# Autodesk Inventor assembly: driver station
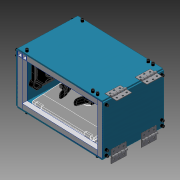
[picture p0: Inventor's stored thumbnail of the model, 180x180]
Saved by Autodesk Inventor 2015 (Build 190159000, 159)
## iProperties
Created: 2015-07-04
Part Number: driver station
Document SubType Name: Assembly
Designer: tsayman
Author: tsayman
## Documents named in this file (15)
- C:\Users\Owner\Documents\GrabCAD\Driver Station\driver station.iam
- C:\Users\Owner\Documents\GrabCAD\Driver Station\Part1.ipt
- C:\Users\Owner\Documents\GrabCAD\Driver Station\Part2.ipt
- C:\Users\Owner\Documents\GrabCAD\Driver Station\Part3.ipt
- C:\Users\Owner\Documents\GrabCAD\Driver Station\Part4.ipt
- C:\Users\Owner\Documents\GrabCAD\Driver Station\Part5.ipt
- C:\Users\Owner\Documents\GrabCAD\Driver Station\Imported Components\Assembly1.iam
- C:\Users\Owner\Documents\GrabCAD\Driver Station\Part6.ipt
- C:\Users\Owner\Documents\GrabCAD\Driver Station\Part7.ipt
- C:\Users\Owner\Documents\GrabCAD\Driver Station\Part8.ipt
- C:\Users\Owner\Documents\GrabCAD\Driver Station\buttonbox standin.ipt
- C:\Users\Owner\Documents\GrabCAD\Driver Station\logitech joystick.ipt
- C:\Users\Owner\Documents\GrabCAD\Driver Station\laptopstandin.ipt
- C:\Users\Owner\Documents\GrabCAD\Driver Station\finalhinge.ipt
- C:\Users\Owner\Documents\GrabCAD\Driver Station\bumper.ipt
## Components (46 placed, 20 different names)
1. bar1 — Mate:12, Flush:19, Flush:20
2. bar 2 — Flush:23, Mate:14, Flush:24
3. bar3 — Flush:21, Flush:22, Mate:13
4. bar4 — Mate:11, Flush:17, Flush:18
5. bar5 — Mate:9, Flush:12, Flush:13
6. bar6 — Mate:6, Flush:6, Flush:7
7. bar7 — Mate:8, Flush:10, Flush:11
8. bar8 — Flush:15, Mate:10, Flush:16
9. bar9 — Mate:3, Flush:4, Flush:14
10. bar10 — Mate:7, Flush:8, Flush:9
11. laptop asm [sub-assembly] — Mate:18
12. left panel — Mate:1, Flush:1, Mate:12, Flush:19, Flush:20, Flush:21, Flush:22, Mate:13, Flush:23, Mate:14, Flush:24, Mate:16, Flush:31, Flush:32, Angle:3, Flush:45, Flush:46, Mate:40, Mate:41, Mate:42, Mate:43, Mate:44, Mate:57, Mate:58, Mate:59, Mate:60, Mate:61
13. bottom pannel — Mate:1, Flush:1, Mate:2, Flush:3, Mate:3, Flush:4, Flush:14, Flush:15, Mate:10, Flush:16, Mate:17, Flush:33, Flush:34, Mate:18, Angle:1, Angle:3, Mate:23, Mate:24, Flush:35, Flush:36, Mate:36, Mate:38, Mate:39, Mate:55, Mate:56, Mate:64, Mate:65, Mate:66
14. top pannel — Flush:5, Mate:4, Mate:6, Flush:6, Flush:7, Mate:7, Flush:8, Flush:9, Mate:8, Flush:10, Flush:11, Rigid:2, Angle:2, Mate:19, Mate:20, Flush:39, Flush:40, Flush:41, Flush:42, Mate:25, Mate:26, Mate:27, Mate:28, Mate:29, Mate:30, Mate:45, Mate:46, Mate:47, Mate:48, Mate:49, Mate:50
15. right pannel — Mate:2, Flush:3, Flush:5, Mate:4, Mate:9, Flush:12, Flush:13, Mate:11, Flush:17, Flush:18, Rigid:1, Angle:1, Angle:2, Mate:21, Mate:22, Flush:37, Flush:38, Flush:43, Flush:44, Mate:31, Mate:32, Mate:33, Mate:34, Mate:35, Mate:51, Mate:52, Mate:53, Mate:54, Mate:62, Mate:63
16. buttonbox standin:1 — Rigid:2
17. logitech joystick:1 — Rigid:1
18. logitech joystick:2 — Mate:16, Flush:31, Flush:32
19. laptopstandin:1 — Mate:17, Flush:33, Flush:34
20. finalhinge:1 — Mate:19, Flush:40, Flush:42
21. finalhinge:2 — Mate:20, Flush:39, Flush:41
22. finalhinge:3 — Mate:22, Flush:38, Flush:43
23. finalhinge:4 — Mate:21, Flush:37, Flush:44
24. finalhinge:5 — Mate:24, Flush:36, Flush:45
25. finalhinge:6 — Mate:23, Flush:35, Flush:46
26. bumper:1 — Mate:39, Mate:66
27. bumper:2 — Mate:40, Mate:59
28. bumper:3 — Mate:64, Mate:65
29. bumper:4 — Mate:36, Mate:55
30. bumper:5 — Mate:38, Mate:56
31. bumper:6 — Mate:35
32. bumper:7 — Mate:34, Mate:52
33. bumper:8 — Mate:33, Mate:54
34. bumper:9 — Mate:41, Mate:58
35. bumper:10 — Mate:42, Mate:61
36. bumper:11 — Mate:43, Mate:60
37. bumper:12 — Mate:44, Mate:57
38. bumper:13 — Mate:32, Mate:53
39. bumper:14 — Mate:31, Mate:51
40. bumper:15 — Mate:30, Mate:49
41. bumper:16 — Mate:29, Mate:50
42. bumper:17 — Mate:27, Mate:46
43. bumper:18 — Mate:28, Mate:45
44. bumper:19 — Mate:26, Mate:48
45. bumper:20 — Mate:25, Mate:47
46. bumper:21 — Mate:62, Mate:63
## Relationships (107: Mate 63, Flush 39, Angle 3, WeldJoint 2)
- Mate:1: left panel ↔ bottom pannel
- Flush:1: left panel ↔ bottom pannel
- Mate:2: bottom pannel ↔ right pannel
- Flush:3: bottom pannel ↔ right pannel
- Mate:3: bar9 ↔ bottom pannel
- Flush:4: bar9 ↔ bottom pannel
- Flush:5: top pannel ↔ right pannel
- Mate:4: top pannel ↔ right pannel
- Mate:6: bar6 ↔ top pannel
- Flush:6 (25.4 mm): bar6 ↔ top pannel
- Flush:7: bar6 ↔ top pannel
- Mate:7: bar10 ↔ top pannel
- Flush:8: bar10 ↔ top pannel
- Flush:9 (50.8 mm): bar10 ↔ top pannel
- Mate:8: bar7 ↔ top pannel
- Flush:10: bar7 ↔ top pannel
- Flush:11 (50.8 mm): bar7 ↔ top pannel
- Mate:9: bar5 ↔ right pannel
- Flush:12: bar5 ↔ right pannel
- Flush:13: bar5 ↔ right pannel
- Flush:14 (25.4 mm): bar9 ↔ bottom pannel
- Flush:15: bar8 ↔ bottom pannel
- Mate:10: bar8 ↔ bottom pannel
- Flush:16 (25.4 mm): bar8 ↔ bottom pannel
- Mate:11: bar4 ↔ right pannel
- Flush:17: bar4 ↔ right pannel
- Flush:18: bar4 ↔ right pannel
- Mate:12: bar1 ↔ left panel
- Flush:19: bar1 ↔ left panel
- Flush:20: bar1 ↔ left panel
- Flush:21: bar3 ↔ left panel
- Flush:22: bar3 ↔ left panel
- Mate:13: bar3 ↔ left panel
- Flush:23: bar 2 ↔ left panel
- Mate:14: bar 2 ↔ left panel
- Flush:24: bar 2 ↔ left panel
- Mate:16: left panel ↔ logitech joystick:2
- Flush:31 (50.8 mm): left panel ↔ logitech joystick:2
- Flush:32 (63.5 mm): left panel ↔ logitech joystick:2
- Rigid:1 [WeldJoint] (12.7 mm): right pannel ↔ logitech joystick:1
- Rigid:2 [WeldJoint]: top pannel ↔ buttonbox standin:1
- Mate:17: bottom pannel ↔ laptopstandin:1
- Flush:33 (38.1 mm): bottom pannel ↔ laptopstandin:1
- Flush:34 (60.325 mm): bottom pannel ↔ laptopstandin:1
- Mate:18: laptop asm ↔ bottom pannel
- Angle:1 (90 deg): bottom pannel ↔ right pannel
- Angle:2 (90 deg): top pannel ↔ right pannel
- Angle:3 (90 deg): left panel ↔ bottom pannel
- Mate:19: top pannel ↔ finalhinge:1
- Mate:20: top pannel ↔ finalhinge:2
- Mate:21: right pannel ↔ finalhinge:4
- Mate:22: right pannel ↔ finalhinge:3
- Mate:23: bottom pannel ↔ finalhinge:6
- Mate:24: bottom pannel ↔ finalhinge:5
- Flush:35 (-38.1 mm): bottom pannel ↔ finalhinge:6
- Flush:36 (-38.1 mm): bottom pannel ↔ finalhinge:5
- Flush:37 (-38.1 mm): right pannel ↔ finalhinge:4
- Flush:38 (-38.1 mm): right pannel ↔ finalhinge:3
- Flush:39 (-38.1 mm): top pannel ↔ finalhinge:2
- Flush:40 (-38.1 mm): top pannel ↔ finalhinge:1
- Flush:41 (38.1 mm): top pannel ↔ finalhinge:2
- Flush:42 (38.1 mm): top pannel ↔ finalhinge:1
- Flush:43 (38.1 mm): right pannel ↔ finalhinge:3
- Flush:44 (38.1 mm): right pannel ↔ finalhinge:4
- Flush:45 (38.1 mm): left panel ↔ finalhinge:5
- Flush:46 (38.1 mm): left panel ↔ finalhinge:6
- Mate:25: top pannel ↔ bumper:20
- Mate:26: top pannel ↔ bumper:19
- Mate:27: top pannel ↔ bumper:17
- Mate:28: top pannel ↔ bumper:18
- Mate:29: top pannel ↔ bumper:16
- Mate:30: top pannel ↔ bumper:15
- Mate:31: right pannel ↔ bumper:14
- Mate:32: right pannel ↔ bumper:13
- Mate:33: right pannel ↔ bumper:8
- Mate:34: right pannel ↔ bumper:7
- Mate:35: right pannel ↔ bumper:6
- Mate:36: bottom pannel ↔ bumper:4
- Mate:38: bottom pannel ↔ bumper:5
- Mate:39: bottom pannel ↔ bumper:1
- Mate:40: left panel ↔ bumper:2
- Mate:41: left panel ↔ bumper:9
- Mate:42: left panel ↔ bumper:10
- Mate:43: left panel ↔ bumper:11
- Mate:44: left panel ↔ bumper:12
- Mate:45: top pannel ↔ bumper:18
- Mate:46: top pannel ↔ bumper:17
- Mate:47: top pannel ↔ bumper:20
- Mate:48: top pannel ↔ bumper:19
- Mate:49: top pannel ↔ bumper:15
- Mate:50: top pannel ↔ bumper:16
- Mate:51: right pannel ↔ bumper:14
- Mate:52: right pannel ↔ bumper:7
- Mate:53: right pannel ↔ bumper:13
- Mate:54: right pannel ↔ bumper:8
- Mate:55: bottom pannel ↔ bumper:4
- Mate:56: bottom pannel ↔ bumper:5
- Mate:57: left panel ↔ bumper:12
- Mate:58: left panel ↔ bumper:9
- Mate:59: left panel ↔ bumper:2
- Mate:60: left panel ↔ bumper:11
- Mate:61: left panel ↔ bumper:10
- Mate:62: right pannel ↔ bumper:21
- Mate:63: right pannel ↔ bumper:21
- Mate:64: bottom pannel ↔ bumper:3
- Mate:65: bottom pannel ↔ bumper:3
- Mate:66: bottom pannel ↔ bumper:1
